# Autodesk Inventor assembly: Clamping hub 1_4 D shortened clamp
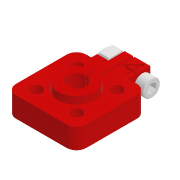
[picture p0: Inventor's stored thumbnail of the model, 180x180]
Saved by Autodesk Inventor 2020 (Build 240168000, 168)
## iProperties
Created: 2019-12-16
Part Number: Clamping hub 1_4 D shortened clamp
Document SubType Name: Assembly
Designer: ball
Author: ball
## Documents named in this file (4)
- C:\FTC\FTC8863CAD\2019 Robot\Generic Parts\Clamping hub 1_4 D shortened clamp.iam
- C:\FTC\FTC8863CAD\2019 Robot\Generic Parts\clamping hub 1_4 D nut wells shortened clamp.ipt
- C:\FTC\FTC8863CAD\StepLibraries\Nuts\6-32 NYLON-INSERT LOCKNUT.ipt
- C:\FTC\FTC8863CAD\StepLibraries\Screws\6-32x.375 SOCKET HEAD CAP SCREW.ipt
## Components (3 placed, 3 different names)
1. clamping hub 1_4 D nut wells shortened clamp:1 — Mate:1, Mate:2, Mate:3, Mate:4, Angle:1
2. 6-32 NYLON-INSERT LOCKNUT:1 — Mate:3, Mate:4, Angle:1
3. 6-32x.375 SOCKET HEAD CAP SCREW:1 — Mate:1, Mate:2
## Relationships (5: Mate 4, Angle 1)
- Mate:1: clamping hub 1_4 D nut wells shortened clamp:1 ↔ 6-32x.375 SOCKET HEAD CAP SCREW:1
- Mate:2: clamping hub 1_4 D nut wells shortened clamp:1 ↔ 6-32x.375 SOCKET HEAD CAP SCREW:1
- Mate:3: clamping hub 1_4 D nut wells shortened clamp:1 ↔ 6-32 NYLON-INSERT LOCKNUT:1
- Mate:4: clamping hub 1_4 D nut wells shortened clamp:1 ↔ 6-32 NYLON-INSERT LOCKNUT:1
- Angle:1 (0 deg): clamping hub 1_4 D nut wells shortened clamp:1 ↔ 6-32 NYLON-INSERT LOCKNUT:1
